# Autodesk Inventor assembly: TempController
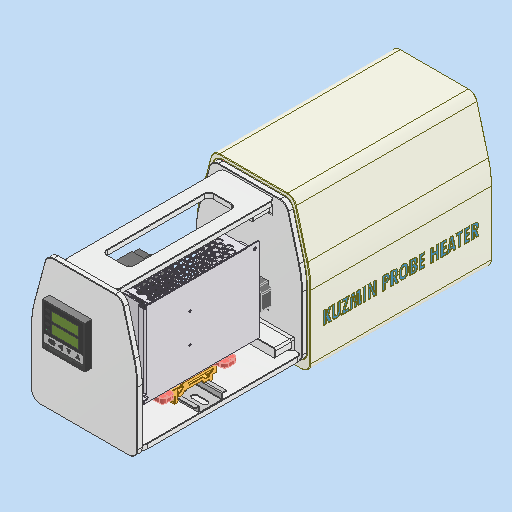
[picture p0: Inventor's stored thumbnail of the model, 512x512]
Saved by Autodesk Inventor 2026 (Build 300175050, 175E)
## iProperties
Created: 2025-05-30
Part Number: TempController
Document SubType Name: Assembly
Designer: kuzmin
Author: kuzmin
## Documents named in this file (13)
- C:\Users\queezz\Dropbox\Drawings\PIHTI\ElectronicsBox\TempController\TempController.iam
- C:\Users\queezz\Dropbox\Drawings\PIHTI\ElectronicsBox\TempController\RKC CONTROLLER.ipt
- C:\Users\queezz\Dropbox\Drawings\PIHTI\ElectronicsBox\TempController\Fuente meanwell LRS-100-12.ipt
- C:\Users\queezz\Dropbox\Drawings\PIHTI\ElectronicsBox\TempController\tc-front-panel.ipt
- C:\Users\queezz\Dropbox\Drawings\PIHTI\ElectronicsBox\TempController\RT-65D-Bracket.ipt
- C:\Users\queezz\Dropbox\Drawings\PIHTI\ElectronicsBox\TempController\Wide Din Clip.ipt
- C:\Users\queezz\Dropbox\Drawings\PIHTI\ElectronicsBox\TempController\DIN-rail-tc.ipt
- C:\Users\queezz\Dropbox\Drawings\PIHTI\ElectronicsBox\TempController\tc-bottom-tray.ipt
- C:\Users\queezz\Dropbox\Drawings\PIHTI\ElectronicsBox\TempController\SSR-on-DIN.iam
- C:\Users\queezz\Dropbox\Drawings\PIHTI\ElectronicsBox\TempController\IEC320 C14 Panel switch.ipt
- C:\Users\queezz\Dropbox\Drawings\PIHTI\ElectronicsBox\TempController\tc-back-panel.ipt
- C:\Users\queezz\Dropbox\Drawings\PIHTI\ElectronicsBox\TempController\tc-case.ipt
- C:\Users\queezz\Dropbox\Drawings\PIHTI\ElectronicsBox\TempController\tc-top-bar.ipt
## Components (12 placed, 12 different names)
1. tc-front-panel:1 — Mate:1, Mate:2, Mate:3, Mate:7, Flush:1, Flush:3, Flush:4, Flush:5, Flush:6, Mate:14, Flush:8
2. RKC CONTROLLER:1 — Mate:1, Mate:2, Mate:3
3. Fuente meanwell LRS-100-12:1 — Rigid:1
4. RT-65D-Bracket:1 — Rigid:1, Rigid:2
5. Wide Din Clip:1 — Rigid:2, Mate:4, Mate:5
6. DIN-rail-tc:1 — Mate:4, Mate:5, Mate:6, Flush:2, Mate:8, Mate:9
7. tc-bottom-tray:1 — Mate:6, Mate:7, Flush:1, Flush:2, Flush:3, Mate:10
8. SSR-on-DIN:1 [sub-assembly] — Mate:8, Mate:9
9. IEC320 C14 Panel switch:1 — Mate:11, Mate:12, Mate:13
10. tc-back-panel:1 — Flush:4, Flush:5, Mate:10, Mate:11, Mate:12, Mate:13, Mate:15, Mate:16, Flush:9
11. tc-case:1 — Flush:6, Mate:14, Mate:15
12. tc-top-bar:1 — Mate:16, Flush:7, Flush:9
## Relationships (27: Mate 16, Flush 9, WeldJoint 2)
- Mate:1: tc-front-panel:1 ↔ RKC CONTROLLER:1
- Mate:2: tc-front-panel:1 ↔ RKC CONTROLLER:1
- Mate:3: tc-front-panel:1 ↔ RKC CONTROLLER:1
- Rigid:1 [WeldJoint]: Fuente meanwell LRS-100-12:1 ↔ RT-65D-Bracket:1
- Rigid:2 [WeldJoint]: RT-65D-Bracket:1 ↔ Wide Din Clip:1
- Mate:4: Wide Din Clip:1 ↔ DIN-rail-tc:1
- Mate:5: Wide Din Clip:1 ↔ DIN-rail-tc:1
- Mate:6: DIN-rail-tc:1 ↔ tc-bottom-tray:1
- Mate:7: tc-front-panel:1 ↔ tc-bottom-tray:1
- Flush:1: tc-front-panel:1 ↔ tc-bottom-tray:1
- Flush:2: DIN-rail-tc:1 ↔ tc-bottom-tray:1
- Flush:3 (5 mm): tc-front-panel:1 ↔ tc-bottom-tray:1
- Mate:8: DIN-rail-tc:1 ↔ SSR-on-DIN:1
- Mate:9: DIN-rail-tc:1 ↔ SSR-on-DIN:1
- Flush:4: tc-front-panel:1 ↔ tc-back-panel:1
- Flush:5: tc-front-panel:1 ↔ tc-back-panel:1
- Mate:10: tc-bottom-tray:1 ↔ tc-back-panel:1
- Mate:11: IEC320 C14 Panel switch:1 ↔ tc-back-panel:1
- Mate:12: IEC320 C14 Panel switch:1 ↔ tc-back-panel:1
- Mate:13: IEC320 C14 Panel switch:1 ↔ tc-back-panel:1
- Flush:6: tc-front-panel:1 ↔ tc-case:1
- Mate:14: tc-front-panel:1 ↔ tc-case:1
- Mate:15: tc-back-panel:1 ↔ tc-case:1
- Mate:16: tc-back-panel:1 ↔ tc-top-bar:1
- Flush:7: tc-top-bar:1
- Flush:8: tc-front-panel:1
- Flush:9 (2 mm): tc-back-panel:1 ↔ tc-top-bar:1
